# Autodesk Inventor assembly: 03-ImageSeparation
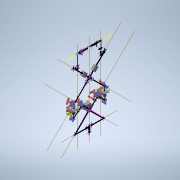
[picture p0: Inventor's stored thumbnail of the model, 180x180]
Saved by Autodesk Inventor 2020 (Build 240168000, 168)
## iProperties
Created: 2016-12-02
Part Number: 03-ImageSeparation
Document SubType Name: Assembly
Designer: map
Author: map
## Documents named in this file (14)
- C:\Users\whgu0532\Documents\4Pi\4Pi-Oxford\03-ImageSeparation.iam
- C:\Users\whgu0532\Documents\4Pi\4Pi-Oxford\__CAVITY_AND_IMAGING_OPTICS__.iam
- C:\Users\whgu0532\Documents\4Pi\4Pi-Oxford\SS100-F3H.ipt
- C:\Users\whgu0532\Documents\4Pi\4Pi-Oxford\FAB-P0019 - Mirror Mount, SS100.ipt
- C:\Users\whgu0532\Documents\4Pi\4Pi-Oxford\Thor LMR1-M Fixed Lens Mt.ipt
- C:\Users\whgu0532\Documents\4Pi\4Pi-Oxford\newfocus_9481.ipt
- C:\Users\whgu0532\Documents\4Pi\R2017\en-US\ISO 4762(1)\DIN EN ISO 4762 - M4 x 40.ipt
- C:\Users\whgu0532\Documents\4Pi\R2017\en-US\ISO 4762(1)\DIN EN ISO 4762 - M4 x 30.ipt
- C:\Users\whgu0532\Documents\4Pi\4Pi-Oxford\ASF-10002 - Mirror Mount, Jogged, SS100.ipt
- C:\Users\whgu0532\Documents\4Pi\4Pi-Oxford\Alignment Assembly after Cavity.iam
- C:\Users\whgu0532\Documents\4Pi\4Pi-Oxford\Owis - 27.160.1212 - Rectangular Aperture 12 mm.ipt
- C:\Users\whgu0532\Documents\4Pi\4Pi-Oxford\ASF-10003 - Aperture Mount WITH SLOT.ipt
- C:\Users\whgu0532\Documents\4Pi\4Pi-Oxford\FAB-P0038 - BS2 Optics Mount.ipt
- C:\Users\whgu0532\Documents\4Pi\4Pi-Oxford\FAB-OX0001.ipt
## Components (31 placed, 18 different names)
1. __CAVITY_AND_IMAGING_OPTICS__:1 [sub-assembly] — Angle:1, Mate:1, Mate:8, Mate:12, Mate:16, Mate:17, Mate:18, Tangent:1, Tangent:2, Mate:25, Mate:26, Mate:31, Mate:35, Angle:3, Mate:36, Mate:37, Mate:38, Mate:39, Mate:40, Mate:41, Angle:4, Angle:5, Angle:6, Angle:7, Angle:8, Angle:9, Mate:44, Mate:47, Angle:11, Mate:48, Mate:49, Angle:12, Angle:14, Angle:15, Mate:56, Angle:16, Mate:57, Angle:17
2. SS100-F3H:1 — Angle:1, Mate:1, Mate:2, Mate:3, Mate:4
3. FAB-P0019 - Mirror Mount, SS100:1 — Mate:2, Mate:3, Mate:4, Angle:2, Flush:1, Flush:2, Flush:3, Symmetry:1, Flush:5, Flush:6, Flush:7, Flush:8, Flush:9, Flush:10, Flush:11, Flush:12, Flush:13
4. SS100-F3H:2 — Mate:5, Mate:8
5. FAB-P0019 - Mirror Mount, SS100:2 — Mate:5, Flush:1, Flush:4, Angle:14
6. SS100-F3H:3 — Mate:9, Mate:11, Mate:12
7. FAB-P0019 - Mirror Mount, SS100:3 — Mate:9, Mate:11, Flush:2, Symmetry:1
8. SS100-F3H:9 — Mate:13, Mate:16
9. FAB-P0019 - Mirror Mount, SS100:4 — Mate:13, Flush:3, Flush:4
10. Thor LMR1-M Fixed Lens Mt:1 — Mate:18, Tangent:1, Mate:19, Mate:20, Mate:52
11. Thor LMR1-M Fixed Lens Mt:2 — Mate:17, Tangent:2, Mate:21, Mate:22
12. newfocus_9481:1 — Mate:24, Mate:27, Mate:50, Mate:51
13. FAB-OX0001 - BS2 Optics Mount:1 — Mate:19, Mate:20, Mate:21, Mate:22, Mate:24, Insert:1, Insert:2, Insert:3
14. DIN EN ISO 4762 M4 x 40:1 — Insert:1
15. DIN EN ISO 4762 M4 x 30:1 — Insert:2, Mate:51
16. DIN EN ISO 4762 M4 x 40:3 — Insert:3
17. SS100-F3H:10 — Mate:28, Mate:29, Mate:30, Mate:31
18. ASF-10002 - Mirror Mount, Jogged, SS100:1 — Mate:28, Mate:29, Mate:30, Flush:5, Symmetry:2, Symmetry:3
19. SS100-F3H:11 — Mate:33, Mate:35
20. ASF-10002 - Mirror Mount, Jogged, SS100:2 — Mate:33, Flush:6, Symmetry:2, Angle:3, Symmetry:3
21. Alignment Assembly after Cavity:Upper1 [sub-assembly] — Flush:8, Mate:36, Angle:9, Angle:12, Flush:20, Flush:21, Mate:67, Mate:68
22. Alignment Assembly after Cavity:Upper2 [sub-assembly] — Flush:7, Mate:37, Angle:8, Mate:68
23. Alignment Assembly after Cavity:Upper3 [sub-assembly] — Flush:9, Mate:38, Angle:7, Flush:18
24. Alignment Assembly after Cavity:Lower1 [sub-assembly] — Flush:10, Mate:39, Angle:5, Angle:15, Flush:20, Mate:69
25. Alignment Assembly after Cavity:Lower2 [sub-assembly] — Flush:11, Flush:13, Mate:40, Angle:4, Mate:69
26. Alignment Assembly after Cavity:Lower3 [sub-assembly] — Flush:12, Mate:41, Angle:6
27. Owis - 27.160.1212 - Rectangular Aperture 12 mm:1 — Mate:44, Mate:56, Angle:16, Mate:65, Mate:66
28. ASF-10003 - Aperture Mount WITH SLOT:1 — Flush:21, Flush:22, Mate:65, Mate:66, Mate:67
29. Owis - 27.160.1212 - Rectangular Aperture 12 mm:2 — Mate:47, Angle:11, Mate:57, Mate:58, Mate:59, Mate:60
30. ASF-10003 - Aperture Mount WITH SLOT:2 — Mate:58, Mate:59, Flush:22, Angle:17, Mate:60
31. FAB-OX0001:1 — Flush:18, Mate:52
## Relationships (97: Mate 57, Flush 17, Angle 15, Symmetry 3, Insert 3, Tangent 2)
- Angle:1 (0 deg): __CAVITY_AND_IMAGING_OPTICS__:1 ↔ SS100-F3H:1
- Mate:1: __CAVITY_AND_IMAGING_OPTICS__:1 ↔ SS100-F3H:1
- Mate:2: SS100-F3H:1 ↔ FAB-P0019 - Mirror Mount, SS100:1
- Mate:3: SS100-F3H:1 ↔ FAB-P0019 - Mirror Mount, SS100:1
- Mate:4: SS100-F3H:1 ↔ FAB-P0019 - Mirror Mount, SS100:1
- Angle:2 (180 deg): FAB-P0019 - Mirror Mount, SS100:1
- Mate:5: SS100-F3H:2 ↔ FAB-P0019 - Mirror Mount, SS100:2
- [Mate]: SS100-F3H:2 ↔ FAB-P0019 - Mirror Mount, SS100:2
- [Mate]: SS100-F3H:2 ↔ FAB-P0019 - Mirror Mount, SS100:2
- Mate:8: __CAVITY_AND_IMAGING_OPTICS__:1 ↔ SS100-F3H:2
- Flush:1: FAB-P0019 - Mirror Mount, SS100:1 ↔ FAB-P0019 - Mirror Mount, SS100:2
- Mate:9: SS100-F3H:3 ↔ FAB-P0019 - Mirror Mount, SS100:3
- [Mate]: SS100-F3H:3 ↔ FAB-P0019 - Mirror Mount, SS100:3
- Mate:11: SS100-F3H:3 ↔ FAB-P0019 - Mirror Mount, SS100:3
- Flush:2: FAB-P0019 - Mirror Mount, SS100:1 ↔ FAB-P0019 - Mirror Mount, SS100:3
- Mate:12: __CAVITY_AND_IMAGING_OPTICS__:1 ↔ SS100-F3H:3
- Mate:13: SS100-F3H:9 ↔ FAB-P0019 - Mirror Mount, SS100:4
- [Mate]: SS100-F3H:9 ↔ FAB-P0019 - Mirror Mount, SS100:4
- [Mate]: SS100-F3H:9 ↔ FAB-P0019 - Mirror Mount, SS100:4
- Flush:3: FAB-P0019 - Mirror Mount, SS100:1 ↔ FAB-P0019 - Mirror Mount, SS100:4
- Mate:16: __CAVITY_AND_IMAGING_OPTICS__:1 ↔ SS100-F3H:9
- Flush:4: FAB-P0019 - Mirror Mount, SS100:2 ↔ FAB-P0019 - Mirror Mount, SS100:4
- Symmetry:1: FAB-P0019 - Mirror Mount, SS100:1 ↔ FAB-P0019 - Mirror Mount, SS100:3
- Mate:17: __CAVITY_AND_IMAGING_OPTICS__:1 ↔ Thor LMR1-M Fixed Lens Mt:2
- Mate:18: __CAVITY_AND_IMAGING_OPTICS__:1 ↔ Thor LMR1-M Fixed Lens Mt:1
- Tangent:1: __CAVITY_AND_IMAGING_OPTICS__:1 ↔ Thor LMR1-M Fixed Lens Mt:1
- Tangent:2: __CAVITY_AND_IMAGING_OPTICS__:1 ↔ Thor LMR1-M Fixed Lens Mt:2
- Mate:19: Thor LMR1-M Fixed Lens Mt:1 ↔ FAB-OX0001 - BS2 Optics Mount:1
- Mate:20: Thor LMR1-M Fixed Lens Mt:1 ↔ FAB-OX0001 - BS2 Optics Mount:1
- Mate:21: Thor LMR1-M Fixed Lens Mt:2 ↔ FAB-OX0001 - BS2 Optics Mount:1
- Mate:22: Thor LMR1-M Fixed Lens Mt:2 ↔ FAB-OX0001 - BS2 Optics Mount:1
- Mate:24: newfocus_9481:1 ↔ FAB-OX0001 - BS2 Optics Mount:1
- Mate:25: __CAVITY_AND_IMAGING_OPTICS__:1
- Mate:26: __CAVITY_AND_IMAGING_OPTICS__:1
- Mate:27: newfocus_9481:1
- Insert:1: FAB-OX0001 - BS2 Optics Mount:1 ↔ DIN EN ISO 4762 M4 x 40:1
- Insert:2: FAB-OX0001 - BS2 Optics Mount:1 ↔ DIN EN ISO 4762 M4 x 30:1
- Insert:3: FAB-OX0001 - BS2 Optics Mount:1 ↔ DIN EN ISO 4762 M4 x 40:3
- Mate:28: SS100-F3H:10 ↔ ASF-10002 - Mirror Mount, Jogged, SS100:1
- Mate:29: SS100-F3H:10 ↔ ASF-10002 - Mirror Mount, Jogged, SS100:1
- Mate:30: SS100-F3H:10 ↔ ASF-10002 - Mirror Mount, Jogged, SS100:1
- Flush:5: FAB-P0019 - Mirror Mount, SS100:1 ↔ ASF-10002 - Mirror Mount, Jogged, SS100:1
- Mate:31: __CAVITY_AND_IMAGING_OPTICS__:1 ↔ SS100-F3H:10
- [Mate]: SS100-F3H:11 ↔ ASF-10002 - Mirror Mount, Jogged, SS100:2
- Mate:33: SS100-F3H:11 ↔ ASF-10002 - Mirror Mount, Jogged, SS100:2
- [Mate]: SS100-F3H:11 ↔ ASF-10002 - Mirror Mount, Jogged, SS100:2
- Mate:35: __CAVITY_AND_IMAGING_OPTICS__:1 ↔ SS100-F3H:11
- Flush:6: FAB-P0019 - Mirror Mount, SS100:1 ↔ ASF-10002 - Mirror Mount, Jogged, SS100:2
- Symmetry:2: ASF-10002 - Mirror Mount, Jogged, SS100:1 ↔ ASF-10002 - Mirror Mount, Jogged, SS100:2
- Angle:3 (0 deg): __CAVITY_AND_IMAGING_OPTICS__:1 ↔ ASF-10002 - Mirror Mount, Jogged, SS100:2
- Flush:7: FAB-P0019 - Mirror Mount, SS100:1 ↔ Alignment Assembly after Cavity:Upper2
- Flush:8: FAB-P0019 - Mirror Mount, SS100:1 ↔ Alignment Assembly after Cavity:Upper1
- Flush:9: FAB-P0019 - Mirror Mount, SS100:1 ↔ Alignment Assembly after Cavity:Upper3
- Flush:10: FAB-P0019 - Mirror Mount, SS100:1 ↔ Alignment Assembly after Cavity:Lower1
- Flush:11: FAB-P0019 - Mirror Mount, SS100:1 ↔ Alignment Assembly after Cavity:Lower2
- Flush:12: FAB-P0019 - Mirror Mount, SS100:1 ↔ Alignment Assembly after Cavity:Lower3
- Flush:13: FAB-P0019 - Mirror Mount, SS100:1 ↔ Alignment Assembly after Cavity:Lower2
- Mate:36: __CAVITY_AND_IMAGING_OPTICS__:1 ↔ Alignment Assembly after Cavity:Upper1
- Mate:37: __CAVITY_AND_IMAGING_OPTICS__:1 ↔ Alignment Assembly after Cavity:Upper2
- Mate:38: __CAVITY_AND_IMAGING_OPTICS__:1 ↔ Alignment Assembly after Cavity:Upper3
- Mate:39: __CAVITY_AND_IMAGING_OPTICS__:1 ↔ Alignment Assembly after Cavity:Lower1
- Mate:40: __CAVITY_AND_IMAGING_OPTICS__:1 ↔ Alignment Assembly after Cavity:Lower2
- Mate:41: __CAVITY_AND_IMAGING_OPTICS__:1 ↔ Alignment Assembly after Cavity:Lower3
- Angle:4 (0 deg): __CAVITY_AND_IMAGING_OPTICS__:1 ↔ Alignment Assembly after Cavity:Lower2
- Angle:5 (1.34 deg): __CAVITY_AND_IMAGING_OPTICS__:1 ↔ Alignment Assembly after Cavity:Lower1
- Angle:6 (0 deg): __CAVITY_AND_IMAGING_OPTICS__:1 ↔ Alignment Assembly after Cavity:Lower3
- Angle:7 (0 deg): __CAVITY_AND_IMAGING_OPTICS__:1 ↔ Alignment Assembly after Cavity:Upper3
- Angle:8 (0 deg): __CAVITY_AND_IMAGING_OPTICS__:1 ↔ Alignment Assembly after Cavity:Upper2
- Angle:9 (2.57 deg): __CAVITY_AND_IMAGING_OPTICS__:1 ↔ Alignment Assembly after Cavity:Upper1
- Mate:44: __CAVITY_AND_IMAGING_OPTICS__:1 ↔ Owis - 27.160.1212 - Rectangular Aperture 12 mm:1
- Mate:47: __CAVITY_AND_IMAGING_OPTICS__:1 ↔ Owis - 27.160.1212 - Rectangular Aperture 12 mm:2
- Angle:11 (0.98 deg): __CAVITY_AND_IMAGING_OPTICS__:1 ↔ Owis - 27.160.1212 - Rectangular Aperture 12 mm:2
- Mate:48: __CAVITY_AND_IMAGING_OPTICS__:1
- Mate:49: __CAVITY_AND_IMAGING_OPTICS__:1
- Mate:50: newfocus_9481:1
- Flush:18: Alignment Assembly after Cavity:Upper3 ↔ FAB-OX0001:1
- Mate:51: newfocus_9481:1 ↔ DIN EN ISO 4762 M4 x 30:1
- Mate:52: Thor LMR1-M Fixed Lens Mt:1 ↔ FAB-OX0001:1
- Angle:12 (90 deg): __CAVITY_AND_IMAGING_OPTICS__:1 ↔ Alignment Assembly after Cavity:Upper1
- Angle:14 (90 deg): __CAVITY_AND_IMAGING_OPTICS__:1 ↔ FAB-P0019 - Mirror Mount, SS100:2
- Angle:15 (90 deg): __CAVITY_AND_IMAGING_OPTICS__:1 ↔ Alignment Assembly after Cavity:Lower1
- Flush:20: Alignment Assembly after Cavity:Upper1 ↔ Alignment Assembly after Cavity:Lower1
- Symmetry:3: ASF-10002 - Mirror Mount, Jogged, SS100:1 ↔ ASF-10002 - Mirror Mount, Jogged, SS100:2
- Flush:21: Alignment Assembly after Cavity:Upper1 ↔ ASF-10003 - Aperture Mount WITH SLOT:1
- Mate:56: __CAVITY_AND_IMAGING_OPTICS__:1 ↔ Owis - 27.160.1212 - Rectangular Aperture 12 mm:1
- Angle:16 (0 deg): __CAVITY_AND_IMAGING_OPTICS__:1 ↔ Owis - 27.160.1212 - Rectangular Aperture 12 mm:1
- Mate:57: __CAVITY_AND_IMAGING_OPTICS__:1 ↔ Owis - 27.160.1212 - Rectangular Aperture 12 mm:2
- Mate:58: Owis - 27.160.1212 - Rectangular Aperture 12 mm:2 ↔ ASF-10003 - Aperture Mount WITH SLOT:2
- Mate:59: Owis - 27.160.1212 - Rectangular Aperture 12 mm:2 ↔ ASF-10003 - Aperture Mount WITH SLOT:2
- Flush:22: ASF-10003 - Aperture Mount WITH SLOT:1 ↔ ASF-10003 - Aperture Mount WITH SLOT:2
- Angle:17 (90 deg): __CAVITY_AND_IMAGING_OPTICS__:1 ↔ ASF-10003 - Aperture Mount WITH SLOT:2
- Mate:60: Owis - 27.160.1212 - Rectangular Aperture 12 mm:2 ↔ ASF-10003 - Aperture Mount WITH SLOT:2
- Mate:65: Owis - 27.160.1212 - Rectangular Aperture 12 mm:1 ↔ ASF-10003 - Aperture Mount WITH SLOT:1
- Mate:66: Owis - 27.160.1212 - Rectangular Aperture 12 mm:1 ↔ ASF-10003 - Aperture Mount WITH SLOT:1
- Mate:67 (18 mm): Alignment Assembly after Cavity:Upper1 ↔ ASF-10003 - Aperture Mount WITH SLOT:1
- Mate:68 (2 mm): Alignment Assembly after Cavity:Upper1 ↔ Alignment Assembly after Cavity:Upper2
- Mate:69 (2 mm): Alignment Assembly after Cavity:Lower1 ↔ Alignment Assembly after Cavity:Lower2
## Named parameters: d15_d10 = 0.2 mm, d16_d11 = 0 mm, d17_d12 = 0 mm, d18_d13 = 0 mm, d19_d9 = 0 mm, d29_d10 = 0.2 mm, d30_d11 = 0 mm, d31_d12 = 0 mm, d32_d13 = 0 mm, d33_d9 = 0 mm, d40_d38 = 0 mm, d41_d39 = 0 mm, d42_d29_d10 = 0.2 mm, d43_d30_d11 = 0 mm, d44_d31_d12 = 0 mm, d45_d32_d13 = 0 mm, d46_d33_d9 = 0 mm, d88_d77 = 0 mm, d89_d78 = 0.2 mm, d90_d79 = 0 mm, d91_d80 = 0 mm, d92_d81 = 0 mm, d93_d82 = 0 mm, d94_d83 = 0 mm, IrisAngleTol = 1.5 deg
